# Autodesk Inventor assembly: linac_lower_ax_mount_2-asm
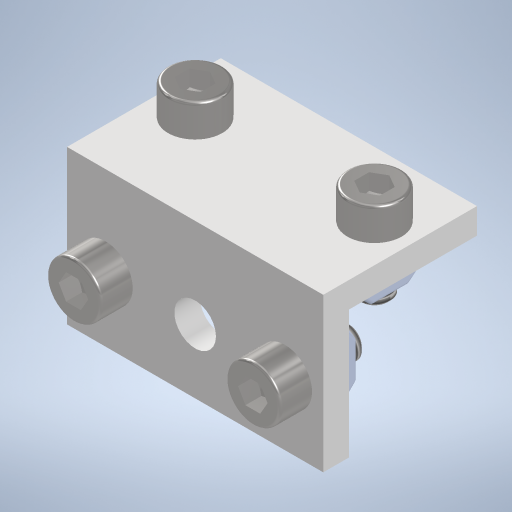
[picture p0: Inventor's stored thumbnail of the model, 512x512]
Saved by Autodesk Inventor 2024 (Build 280153000, 153)
## iProperties
Created: 2025-12-26
Part Number: linac_lower_ax_mount_2-asm
Document SubType Name: Assembly
Designer: schar
Author: schar
## Documents named in this file (4)
- C:\Users\schar\Desktop\projectBlueprint\AMSTS\hardware\linac_lower_ax_mount_2-asm.iam
- C:\Users\schar\Desktop\projectBlueprint\AMSTS\hardware\linac_lower_ax_mount_2.ipt
- C:\Users\schar\Desktop\projectBlueprint\AMSTS\hardware\tnut_m5_2020.ipt
- C:\Users\schar\Documents\Inventor\Content Center Files\R2024\en-US\ISO 4762(1)\DIN EN ISO 4762 - M5 x 10.ipt
## Components (9 placed, 3 different names)
1. linac_lower_ax_mount_2:1 — Rigid:3, Rigid:4, Rigid:1, Rigid:2, Mate:1, Mate:2, Mate:3, Mate:4
2. tnut_m5_2020:1 — Rigid:3, Mate:5
3. tnut_m5_2020:2 — Rigid:4, Mate:6
4. tnut_m5_2020:3 — Rigid:1, Mate:7
5. tnut_m5_2020:4 — Rigid:2, Mate:8
6. DIN EN ISO 4762 M5 x 10:1 — Mate:3, Mate:6
7. DIN EN ISO 4762 M5 x 10:2 — Mate:4, Mate:5
8. DIN EN ISO 4762 M5 x 10:3 — Mate:1, Mate:8
9. DIN EN ISO 4762 M5 x 10:4 — Mate:2, Mate:7
## Relationships (12: Mate 8, WeldJoint 4)
- Rigid:3 [WeldJoint] (0.159 mm): linac_lower_ax_mount_2:1 ↔ tnut_m5_2020:1
- Rigid:4 [WeldJoint] (0.159 mm): linac_lower_ax_mount_2:1 ↔ tnut_m5_2020:2
- Rigid:1 [WeldJoint] (0.159 mm): linac_lower_ax_mount_2:1 ↔ tnut_m5_2020:3
- Rigid:2 [WeldJoint] (0.159 mm): linac_lower_ax_mount_2:1 ↔ tnut_m5_2020:4
- Mate:1: linac_lower_ax_mount_2:1 ↔ DIN EN ISO 4762 M5 x 10:3
- Mate:2: linac_lower_ax_mount_2:1 ↔ DIN EN ISO 4762 M5 x 10:4
- Mate:3: linac_lower_ax_mount_2:1 ↔ DIN EN ISO 4762 M5 x 10:1
- Mate:4: linac_lower_ax_mount_2:1 ↔ DIN EN ISO 4762 M5 x 10:2
- Mate:5: tnut_m5_2020:1 ↔ DIN EN ISO 4762 M5 x 10:2
- Mate:6: tnut_m5_2020:2 ↔ DIN EN ISO 4762 M5 x 10:1
- Mate:7: tnut_m5_2020:3 ↔ DIN EN ISO 4762 M5 x 10:4
- Mate:8: tnut_m5_2020:4 ↔ DIN EN ISO 4762 M5 x 10:3
